# Autodesk Inventor assembly: hipjoint_toleg_right
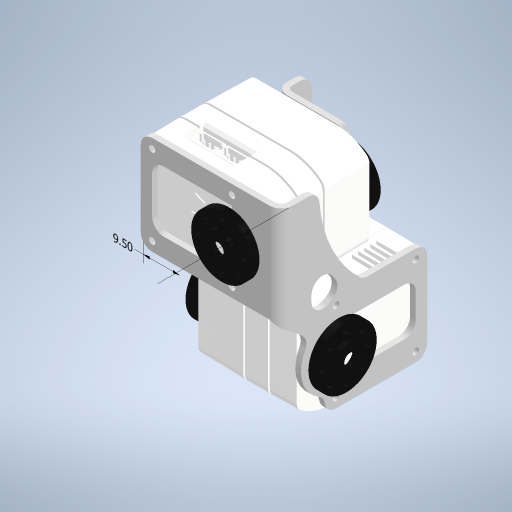
[picture p0: Inventor's stored thumbnail of the model, 512x512]
Saved by Autodesk Inventor 2024.1 (Build 281209000, 209)
## iProperties
Created: 2024-10-09
Part Number: hipjoint_toleg_right
Document SubType Name: Assembly
Designer: hibik
Author: hibik
## Documents named in this file (5)
- C:\Users\hibik\Documents\Robomech\HR\Eglantyne\hard\under_body\hipjoint_toleg_right.iam
- C:\Users\hibik\Documents\Robomech\HR\Eglantyne\hard\needed_model\KRS3300モータ.ipt
- C:\Users\hibik\Documents\Robomech\HR\Eglantyne\hard\under_body\hipjoint_toleg_upper_right.ipt
- C:\Users\hibik\Documents\Robomech\HR\Eglantyne\hard\under_body\hipjoint_toleg_under_right.ipt
- C:\Users\hibik\Documents\Robomech\HR\Eglantyne\hard\needed_model\KRS3300サーボホーン.ipt
## Components (8 placed, 4 different names)
1. KRS3300モータ:1 — 挿入:1, 角度:1, 挿入:4, 挿入:5
2. hipjoint_toleg_upper_right:1 — 挿入:1, 角度:1, 挿入:2, 角度:2
3. KRS3300モータ:2 — 挿入:2, 角度:2, 挿入:3, 角度:3, 挿入:6, 挿入:7
4. hipjoint_toleg_under_right:1 — 挿入:3, 角度:3
5. KRS3300サーボホーン:1 — 挿入:5
6. KRS3300サーボホーン:2 — 挿入:4
7. KRS3300サーボホーン:3 — 挿入:6
8. KRS3300サーボホーン:4 — 挿入:7
## Relationships (10: Insert 7, Angle 3)
- 挿入:1 [Insert]: KRS3300モータ:1 ↔ hipjoint_toleg_upper_right:1
- 角度:1 [Angle] (0 deg): KRS3300モータ:1 ↔ hipjoint_toleg_upper_right:1
- 挿入:2 [Insert]: hipjoint_toleg_upper_right:1 ↔ KRS3300モータ:2
- 角度:2 [Angle] (0 deg): hipjoint_toleg_upper_right:1 ↔ KRS3300モータ:2
- 挿入:3 [Insert]: KRS3300モータ:2 ↔ hipjoint_toleg_under_right:1
- 角度:3 [Angle] (0 deg): KRS3300モータ:2 ↔ hipjoint_toleg_under_right:1
- 挿入:4 [Insert]: KRS3300モータ:1 ↔ KRS3300サーボホーン:2
- 挿入:5 [Insert]: KRS3300モータ:1 ↔ KRS3300サーボホーン:1
- 挿入:6 [Insert]: KRS3300モータ:2 ↔ KRS3300サーボホーン:3
- 挿入:7 [Insert]: KRS3300モータ:2 ↔ KRS3300サーボホーン:4
